# Autodesk Inventor assembly: 自動販賣機3.3
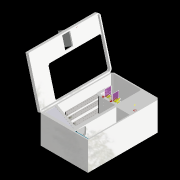
[picture p0: Inventor's stored thumbnail of the model, 180x180]
Saved by Autodesk Inventor 2020 (Build 240168000, 168)
## iProperties
Created: 2021-04-08
Part Number: 自動販賣機3.3
Document SubType Name: Assembly
Designer: 88690
Author: 88690
## Documents named in this file (25)
- C:\Users\88690\Desktop\自動販賣機\自動販賣機3.3.iam
- C:\Users\88690\Desktop\自動販賣機\上滑軌.ipt
- C:\Users\88690\Desktop\自動販賣機\上滑軌輪.ipt
- C:\Users\88690\Desktop\自動販賣機\下滑軌.ipt
- C:\Users\88690\Desktop\自動販賣機\下滑軌輪.ipt
- C:\Users\88690\Desktop\自動販賣機\本體.ipt
- C:\Users\88690\Desktop\自動販賣機\置物架.ipt
- C:\Users\88690\Desktop\自動販賣機\滾筒.ipt
- C:\Users\88690\Desktop\自動販賣機\蓋.ipt
- C:\Users\88690\Desktop\自動販賣機\鎖點支架.ipt
- C:\Users\88690\Desktop\自動販賣機\下支架右.ipt
- C:\Users\88690\Desktop\自動販賣機\上滑軌右.ipt
- C:\Users\88690\Desktop\自動販賣機\蝸桿支架.ipt
- C:\Users\88690\Desktop\自動販賣機\蝸桿滑塊.ipt
- C:\Users\88690\Desktop\自動販賣機\短蝸桿.ipt
- C:\Users\88690\Desktop\自動販賣機\長蝸桿.ipt
- C:\Users\88690\Desktop\自動販賣機\位移平台.ipt
- C:\Users\88690\Desktop\自動販賣機\取物窗.ipt
- C:\Users\88690\Desktop\自動販賣機\螺旋鉤子.ipt
- C:\Users\88690\Desktop\自動販賣機\螺旋鉤子底座.ipt
- C:\Users\88690\Desktop\自動販賣機\名牌1.ipt
- C:\Users\88690\Desktop\自動販賣機\名牌2.ipt
- C:\Users\88690\Desktop\自動販賣機\模擬商品.ipt
- C:\Users\88690\Desktop\自動販賣機\模擬錢幣.ipt
- C:\Users\88690\Desktop\自動販賣機\商品支架.ipt
## Components (47 placed, 24 different names)
1. 上滑軌:1 — 貼合:41, 貼合:42, 貼合:45, 相切:7, 貼合:183
2. 上滑軌輪:1 — 貼合:41, 貼合:42, 相切:1
3. 下滑軌:1 — 貼合:11, 貼合:12, 貼合:13, 貼合:15, 相切:1, 角度:40
4. 下滑軌輪:1 — 貼合:11, 貼合:12, 相切:7
5. 本體:1 — 齊平:1, 齊平:2, 齊平:3, 貼合:1, 貼合:2, 貼合:3, 貼合:4, 貼合:6, 貼合:7, 貼合:8, 貼合:9, 貼合:75, 貼合:76, 貼合:77, 貼合:78, 貼合:79, 貼合:80, 貼合:81, 貼合:82, 貼合:83, 貼合:84, 貼合:85, 貼合:86, 貼合:88, 貼合:89, 貼合:101, 齊平:23, 角度:1, 旋轉:1, 貼合:167, 角度:34, 貼合:169, 貼合:171, 貼合:172, 齊平:53
6. 置物架:1 — 貼合:45, 貼合:50, 貼合:51, 貼合:111, 貼合:131, 貼合:143, 貼合:144, 貼合:145, 旋轉:2, 旋轉:3, 齊平:53, 角度:40, 貼合:183, 角度:41, 貼合:187, 貼合:218, 貼合:219, 貼合:220, 相切:13, 相切:14, 相切:15
7. 滾筒:1 — 貼合:75, 貼合:76, 齊平:14, 齊平:15, 齊平:16, 齊平:17, 齊平:18, 齊平:19, 齊平:20, 齊平:21, 齊平:22, 角度:12, 旋轉:1, 旋轉:1
8. 蓋:1 — 貼合:101, 齊平:23, 角度:1, 角度:2, 貼合:108, 貼合:164, 角度:34, 角度:35
9. 鎖點支架:1 — 貼合:1, 貼合:2, 貼合:3, 齊平:4, 齊平:5, 齊平:6, 齊平:7, 貼合:5, 貼合:15
10. 鎖點支架:2 — 齊平:5, 齊平:7, 貼合:5, 貼合:13, 貼合:51
11. 鎖點支架:3 — 齊平:4, 齊平:6, 貼合:4
12. 鎖點支架:4 — 齊平:8, 齊平:10, 貼合:9
13. 鎖點支架:5 — 貼合:6, 貼合:7, 貼合:8, 齊平:8, 齊平:9, 齊平:10, 齊平:11, 貼合:10, 貼合:30
14. 鎖點支架:6 — 齊平:9, 齊平:11, 貼合:10, 貼合:28
15. 下支架右:1 — 貼合:26, 貼合:27, 貼合:28, 貼合:30, 相切:2, 貼合:74, 角度:41
16. 下滑軌輪:4 — 貼合:26, 貼合:27, 相切:10
17. 上滑軌右:1 — 貼合:46, 貼合:50, 相切:10, 貼合:186, 貼合:187
18. 上滑軌輪:2 — 貼合:46, 相切:2, 貼合:74, 貼合:186
19. 滾筒:2 — 齊平:14, 貼合:77, 旋轉:1, 旋轉:2, 角度:13
20. 滾筒:3 — 齊平:15, 貼合:78, 旋轉:2, 角度:14, 旋轉:3
21. 滾筒:4 — 齊平:16, 貼合:79, 角度:15, 旋轉:3, 旋轉:4
22. 滾筒:5 — 齊平:17, 貼合:80, 角度:16, 旋轉:4, 旋轉:5
23. 滾筒:6 — 齊平:18, 貼合:81, 角度:18, 旋轉:5, 旋轉:6
24. 滾筒:7 — 齊平:19, 貼合:82, 角度:19, 旋轉:6, 旋轉:7
25. 滾筒:8 — 齊平:20, 貼合:83, 角度:22, 旋轉:7, 旋轉:8
26. 滾筒:9 — 齊平:21, 貼合:84, 角度:20, 旋轉:8, 旋轉:9
27. 滾筒:10 — 齊平:22, 貼合:85, 角度:21, 旋轉:9
28. 蝸桿支架:1 — 貼合:86, 貼合:88, 貼合:89, 貼合:90, 貼合:91, 貼合:92, 貼合:93
29. 蝸桿滑塊:1 — 貼合:90, 貼合:91, 貼合:94, 貼合:95, 貼合:97, 貼合:98, 貼合:99
30. 短蝸桿:1 — 貼合:94, 貼合:95, 旋轉/轉換:1
31. 長蝸桿:1 — 貼合:92, 貼合:93, 角度:23, 旋轉/轉換:1
32. 位移平台:1 — 貼合:97, 貼合:98, 貼合:99, 貼合:167
33. 取物窗:1 — 角度:2, 貼合:108, 貼合:164, 角度:35
34. 螺旋鉤子:1 — 貼合:111, 貼合:112, 貼合:113, 角度:3, 貼合:155, 貼合:191, 貼合:199, 貼合:209
35. 螺旋鉤子底座:1 — 貼合:112, 貼合:113, 貼合:155, 旋轉:2
36. 螺旋鉤子:2 — 貼合:131, 角度:45, 貼合:221, 貼合:222, 貼合:223, 貼合:224, 貼合:225, 貼合:226
37. 螺旋鉤子底座:2 — 旋轉:3, 角度:44
38. 名牌1:1 — 貼合:143, 貼合:144, 角度:24, 齊平:30, 角度:25
39. 名牌2:1 — 貼合:145, 齊平:30, 角度:25
40. 模擬錢幣:1 — 貼合:169, 貼合:171, 貼合:172
41. 模擬商品:2 — 貼合:221, 相切:13, 貼合:222
42. 模擬商品:3 — 貼合:191
43. 模擬商品:12 — 貼合:199
44. 模擬商品:21 — 貼合:209
45. 商品支架:1 — 貼合:218, 貼合:219, 貼合:220
46. 模擬商品:22 — 貼合:223, 貼合:226, 相切:15
47. 模擬商品:23 — 貼合:224, 貼合:225, 相切:14
## Relationships (145: Mate 80, Flush 23, Angle 22, RelateRotation 9, Tangent 7, RevoluteJoint 3, RelateRotateTranslate 1)
- 齊平:1 [Flush]: 本體:1
- 齊平:2 [Flush]: 本體:1
- 齊平:3 [Flush]: 本體:1
- 貼合:1 [Mate] (180 mm): 本體:1 ↔ 鎖點支架:1
- 貼合:2 [Mate]: 本體:1 ↔ 鎖點支架:1
- 貼合:3 [Mate]: 本體:1 ↔ 鎖點支架:1
- 齊平:4 [Flush]: 鎖點支架:1 ↔ 鎖點支架:3
- 齊平:5 [Flush]: 鎖點支架:1 ↔ 鎖點支架:2
- 齊平:6 [Flush]: 鎖點支架:1 ↔ 鎖點支架:3
- 齊平:7 [Flush]: 鎖點支架:1 ↔ 鎖點支架:2
- 貼合:4 [Mate]: 本體:1 ↔ 鎖點支架:3
- 貼合:5 [Mate] (55 mm): 鎖點支架:1 ↔ 鎖點支架:2
- 貼合:6 [Mate]: 本體:1 ↔ 鎖點支架:5
- 貼合:7 [Mate]: 本體:1 ↔ 鎖點支架:5
- 貼合:8 [Mate] (180 mm): 本體:1 ↔ 鎖點支架:5
- 齊平:8 [Flush]: 鎖點支架:4 ↔ 鎖點支架:5
- 齊平:9 [Flush]: 鎖點支架:5 ↔ 鎖點支架:6
- 齊平:10 [Flush]: 鎖點支架:4 ↔ 鎖點支架:5
- 齊平:11 [Flush]: 鎖點支架:5 ↔ 鎖點支架:6
- 貼合:9 [Mate]: 本體:1 ↔ 鎖點支架:4
- 貼合:10 [Mate] (55 mm): 鎖點支架:5 ↔ 鎖點支架:6
- 貼合:11 [Mate]: 下滑軌:1 ↔ 下滑軌輪:1
- 貼合:12 [Mate]: 下滑軌:1 ↔ 下滑軌輪:1
- 貼合:13 [Mate]: 下滑軌:1 ↔ 鎖點支架:2
- 貼合:15 [Mate]: 下滑軌:1 ↔ 鎖點支架:1
- 貼合:26 [Mate]: 下支架右:1 ↔ 下滑軌輪:4
- 貼合:27 [Mate]: 下支架右:1 ↔ 下滑軌輪:4
- 貼合:28 [Mate]: 鎖點支架:6 ↔ 下支架右:1
- 貼合:30 [Mate]: 鎖點支架:5 ↔ 下支架右:1
- 貼合:41 [Mate]: 上滑軌:1 ↔ 上滑軌輪:1
- 貼合:42 [Mate]: 上滑軌:1 ↔ 上滑軌輪:1
- 貼合:45 [Mate]: 上滑軌:1 ↔ 置物架:1
- 貼合:46 [Mate]: 上滑軌右:1 ↔ 上滑軌輪:2
- 貼合:50 [Mate]: 置物架:1 ↔ 上滑軌右:1
- 相切:1 [Tangent]: 上滑軌輪:1 ↔ 下滑軌:1
- 相切:2 [Tangent]: 下支架右:1 ↔ 上滑軌輪:2
- 貼合:51 [Mate]: 置物架:1 ↔ 鎖點支架:2
- 貼合:74 [Mate]: 下支架右:1 ↔ 上滑軌輪:2
- 貼合:75 [Mate]: 本體:1 ↔ 滾筒:1
- 貼合:76 [Mate]: 本體:1 ↔ 滾筒:1
- 齊平:14 [Flush]: 滾筒:1 ↔ 滾筒:2
- 齊平:15 [Flush]: 滾筒:1 ↔ 滾筒:3
- 齊平:16 [Flush]: 滾筒:1 ↔ 滾筒:4
- 齊平:17 [Flush]: 滾筒:1 ↔ 滾筒:5
- 齊平:18 [Flush]: 滾筒:1 ↔ 滾筒:6
- 齊平:19 [Flush]: 滾筒:1 ↔ 滾筒:7
- 齊平:20 [Flush]: 滾筒:1 ↔ 滾筒:8
- 齊平:21 [Flush]: 滾筒:1 ↔ 滾筒:9
- 齊平:22 [Flush]: 滾筒:1 ↔ 滾筒:10
- 貼合:77 [Mate]: 本體:1 ↔ 滾筒:2
- 貼合:78 [Mate]: 本體:1 ↔ 滾筒:3
- 貼合:79 [Mate]: 本體:1 ↔ 滾筒:4
- 貼合:80 [Mate]: 本體:1 ↔ 滾筒:5
- 貼合:81 [Mate]: 本體:1 ↔ 滾筒:6
- 貼合:82 [Mate]: 本體:1 ↔ 滾筒:7
- 貼合:83 [Mate]: 本體:1 ↔ 滾筒:8
- 貼合:84 [Mate]: 本體:1 ↔ 滾筒:9
- 貼合:85 [Mate]: 本體:1 ↔ 滾筒:10
- 貼合:86 [Mate]: 本體:1 ↔ 蝸桿支架:1
- 貼合:88 [Mate]: 本體:1 ↔ 蝸桿支架:1
- 貼合:89 [Mate]: 本體:1 ↔ 蝸桿支架:1
- 貼合:90 [Mate]: 蝸桿支架:1 ↔ 蝸桿滑塊:1
- 貼合:91 [Mate]: 蝸桿支架:1 ↔ 蝸桿滑塊:1
- 貼合:92 [Mate]: 蝸桿支架:1 ↔ 長蝸桿:1
- 貼合:93 [Mate]: 蝸桿支架:1 ↔ 長蝸桿:1
- 貼合:94 [Mate]: 蝸桿滑塊:1 ↔ 短蝸桿:1
- 貼合:95 [Mate]: 蝸桿滑塊:1 ↔ 短蝸桿:1
- 貼合:97 [Mate]: 蝸桿滑塊:1 ↔ 位移平台:1
- 貼合:98 [Mate]: 蝸桿滑塊:1 ↔ 位移平台:1
- 貼合:99 [Mate]: 蝸桿滑塊:1 ↔ 位移平台:1
- 貼合:101 [Mate]: 本體:1 ↔ 蓋:1
- 齊平:23 [Flush]: 本體:1 ↔ 蓋:1
- 角度:1 [Angle] (45 deg): 本體:1 ↔ 蓋:1
- 角度:2 [Angle] (180 deg): 蓋:1 ↔ 取物窗:1
- 貼合:108 [Mate]: 蓋:1 ↔ 取物窗:1
- 貼合:111 [Mate]: 置物架:1 ↔ 螺旋鉤子:1
- 貼合:112 [Mate]: 螺旋鉤子:1 ↔ 螺旋鉤子底座:1
- 貼合:113 [Mate]: 螺旋鉤子:1 ↔ 螺旋鉤子底座:1
- 角度:3 [Angle] (0 deg): 螺旋鉤子:1
- [Mate]: 螺旋鉤子:2 ↔ 螺旋鉤子底座:2
- [Mate]: 螺旋鉤子:2 ↔ 螺旋鉤子底座:2
- 貼合:131 [Mate]: 置物架:1 ↔ 螺旋鉤子:2
- 角度:12 [Angle] (4455 deg): 滾筒:1
- 旋轉:1 [RelateRotation] (1 ul): 滾筒:1 ↔ 滾筒:2
- 旋轉:2 [RelateRotation] (1 ul): 滾筒:2 ↔ 滾筒:3
- 角度:13 [Angle] (135 deg): 滾筒:2
- 角度:14 [Angle] (135 deg): 滾筒:3
- 角度:15 [Angle] (135 deg): 滾筒:4
- 角度:16 [Angle] (135 deg): 滾筒:5
- 角度:18 [Angle] (135 deg): 滾筒:6
- 角度:19 [Angle] (135 deg): 滾筒:7
- 角度:20 [Angle] (135 deg): 滾筒:9
- 角度:21 [Angle] (135 deg): 滾筒:10
- 角度:22 [Angle] (135 deg): 滾筒:8
- 旋轉:3 [RelateRotation] (1 ul): 滾筒:3 ↔ 滾筒:4
- 旋轉:4 [RelateRotation] (1 ul): 滾筒:4 ↔ 滾筒:5
- 旋轉:5 [RelateRotation] (1 ul): 滾筒:5 ↔ 滾筒:6
- 旋轉:6 [RelateRotation] (1 ul): 滾筒:6 ↔ 滾筒:7
- 旋轉:7 [RelateRotation] (1 ul): 滾筒:7 ↔ 滾筒:8
- 旋轉:8 [RelateRotation] (1 ul): 滾筒:8 ↔ 滾筒:9
- 旋轉:9 [RelateRotation] (1 ul): 滾筒:9 ↔ 滾筒:10
- 旋轉:1 [RevoluteJoint]: 本體:1 ↔ 滾筒:1
- 角度:23 [Angle] (0 deg): 長蝸桿:1
- 旋轉/轉換:1 [RelateRotateTranslate] (103.673 mm): 短蝸桿:1 ↔ 長蝸桿:1
- 貼合:143 [Mate]: 置物架:1 ↔ 名牌1:1
- 貼合:144 [Mate]: 置物架:1 ↔ 名牌1:1
- 角度:24 [Angle] (0 deg): 名牌1:1
- 貼合:145 [Mate]: 置物架:1 ↔ 名牌2:1
- 齊平:30 [Flush]: 名牌1:1 ↔ 名牌2:1
- 角度:25 [Angle] (0 deg): 名牌1:1 ↔ 名牌2:1
- 貼合:155 [Mate]: 螺旋鉤子:1 ↔ 螺旋鉤子底座:1
- 旋轉:2 [RevoluteJoint]: 置物架:1 ↔ 螺旋鉤子底座:1
- 旋轉:3 [RevoluteJoint]: 置物架:1 ↔ 螺旋鉤子底座:2
- 貼合:164 [Mate]: 蓋:1 ↔ 取物窗:1
- 貼合:167 [Mate]: 本體:1 ↔ 位移平台:1
- 角度:34 [Angle] (75 deg): 本體:1 ↔ 蓋:1
- 角度:35 [Angle] (135 deg): 蓋:1 ↔ 取物窗:1
- 貼合:169 [Mate] (0.5 mm): 本體:1 ↔ 模擬錢幣:1
- 貼合:171 [Mate]: 本體:1 ↔ 模擬錢幣:1
- 貼合:172 [Mate] (150 mm): 本體:1 ↔ 模擬錢幣:1
- 齊平:53 [Flush] (-390 mm): 本體:1 ↔ 置物架:1
- 角度:40 [Angle] (0 deg): 下滑軌:1 ↔ 置物架:1
- 相切:7 [Tangent]: 上滑軌:1 ↔ 下滑軌輪:1
- 貼合:183 [Mate]: 上滑軌:1 ↔ 置物架:1
- 角度:41 [Angle] (0 deg): 置物架:1 ↔ 下支架右:1
- 相切:10 [Tangent]: 下滑軌輪:4 ↔ 上滑軌右:1
- 貼合:186 [Mate]: 上滑軌右:1 ↔ 上滑軌輪:2
- 貼合:187 [Mate]: 置物架:1 ↔ 上滑軌右:1
- 貼合:191 [Mate]: 螺旋鉤子:1 ↔ 模擬商品:3
- 貼合:199 [Mate]: 螺旋鉤子:1 ↔ 模擬商品:12
- 貼合:209 [Mate]: 螺旋鉤子:1 ↔ 模擬商品:21
- 角度:44 [Angle] (0 deg): 螺旋鉤子底座:2
- 貼合:218 [Mate]: 置物架:1 ↔ 商品支架:1
- 貼合:219 [Mate]: 置物架:1 ↔ 商品支架:1
- 貼合:220 [Mate]: 置物架:1 ↔ 商品支架:1
- 角度:45 [Angle] (180 deg): 螺旋鉤子:2
- 貼合:221 [Mate]: 螺旋鉤子:2 ↔ 模擬商品:2
- 相切:13 [Tangent]: 置物架:1 ↔ 模擬商品:2
- 貼合:222 [Mate]: 螺旋鉤子:2 ↔ 模擬商品:2
- 貼合:223 [Mate]: 螺旋鉤子:2 ↔ 模擬商品:22
- 貼合:224 [Mate]: 螺旋鉤子:2 ↔ 模擬商品:23
- 貼合:225 [Mate]: 螺旋鉤子:2 ↔ 模擬商品:23
- 貼合:226 [Mate]: 螺旋鉤子:2 ↔ 模擬商品:22
- 相切:14 [Tangent]: 置物架:1 ↔ 模擬商品:23
- 相切:15 [Tangent]: 置物架:1 ↔ 模擬商品:22
## Named parameters: d158_d154 = 0 mm, d159_d155 = 0 mm
